# Autodesk Inventor assembly: tire_mold_assm
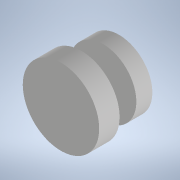
[picture p0: Inventor's stored thumbnail of the model, 180x180]
Saved by Autodesk Inventor 2020 (Build 240168000, 168)
## iProperties
Created: 2020-06-07
Part Number: tire_mold_assm
Document SubType Name: Assembly
Designer: Abhinav Roy
Author: Abhinav Roy
## Documents named in this file (3)
- D:\Mopping_Robot\cad\V1.0\tire_mold_assm.iam
- D:\Mopping_Robot\cad\V1.0\tire_mold_inner.ipt
- D:\Mopping_Robot\cad\V1.0\tire_mold_outer.ipt
## Components (2 placed, 2 different names)
1. tire_mold_inner:1 — Mate:1
2. tire_mold_outer:1 — Mate:1
## Relationships (1: Mate 1)
- Mate:1: tire_mold_inner:1 ↔ tire_mold_outer:1
